# Autodesk Inventor assembly: y_carryage
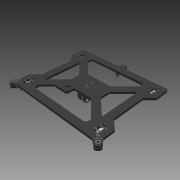
[picture p0: Inventor's stored thumbnail of the model, 180x180]
Saved by Autodesk Inventor 2014 (Build 180170000, 170)
## iProperties
Created: 2014-01-11
Part Number: y_carryage
Document SubType Name: Assembly
Designer: buben
Author: buben
## Documents named in this file (16)
- C:\Users\buben\Documents\GitHub\bacon\inventor files\assemblies\y_carryage.iam
- C:\Users\buben\Documents\GitHub\bacon\inventor files\printer parts\y_carriage.ipt
- C:\Users\buben\Documents\GitHub\bacon\inventor files\3rd party components\linear_bearing_8\Imported Components\LU8MM\LU8MM.iam
- C:\Users\buben\Documents\GitHub\bacon\inventor files\utils\washer_m5.ipt
- C:\Users\buben\Documents\GitHub\bacon\inventor files\utils\washer_m4.ipt
- C:\Users\buben\Documents\GitHub\bacon\inventor files\printer parts\y_carriage_nut_holder_a.ipt
- C:\Users\buben\Documents\GitHub\bacon\inventor files\printer parts\y_carriage_nut_holder_b.ipt
- C:\Users\buben\Documents\Inventor\Content Center Files\R2014\en-US\CSN EN 24032\ISO 4032 - M5CSN EN.ipt
- C:\Users\buben\Documents\Inventor\Content Center Files\R2014\en-US\ISO 7040\ISO 7040 - M4.ipt
- C:\Users\buben\Documents\Inventor\Content Center Files\R2014\en-US\ISO 4762(2)\ISO 4762 - M4 x 25ISO.ipt
- C:\Users\buben\Documents\GitHub\bacon\inventor files\printer parts\y_carriage_belt_mount_bed_holder.ipt
- C:\Users\buben\Documents\GitHub\bacon\inventor files\printer parts\y_carriage_belt_mount.ipt
- C:\Users\buben\Documents\Inventor\Content Center Files\R2014\en-US\ISO 4762(2)\ISO 4762 - M4 x 30ISO.ipt
- C:\Users\buben\Documents\GitHub\bacon\inventor files\utils\y_carryage_bearing_zip_tie.ipt
- C:\Users\buben\Documents\GitHub\bacon\inventor files\utils\y_carryage_nut_holder_b_zip_tie.ipt
- C:\Users\buben\Documents\GitHub\bacon\inventor files\utils\y_carryage_nut_holder_a_zip_tie.ipt
## Components (62 placed, 15 different names)
1. y_carriage:1 — Mate:4, Mate:5, Mate:6, Mate:7, Mate:8, Mate:9, Mate:10, Mate:11, Mate:12, Mate:13, Mate:14, Mate:15, Mate:16, Mate:17, Flush:1, Mate:18, Mate:19, Mate:20, Mate:21, Mate:22, Mate:23, Mate:24, Mate:25, Mate:26, Mate:27, Mate:28, Mate:29, Mate:30, Mate:31, Mate:32, Mate:33, Mate:34, Mate:35, Mate:36, Mate:37, Mate:38, Mate:39, Mate:40, Mate:41, Mate:43, Mate:45, Mate:47, Flush:2, Flush:3, Flush:4, Mate:75, Mate:76, Mate:77, Mate:78, Mate:79, Mate:80, Mate:81, Mate:102, Mate:104, Mate:105, Mate:106, Mate:108, Mate:109, Mate:111, Mate:112, Mate:114, Mate:115, Mate:117, Mate:118, Mate:120, Mate:121, Mate:123, Mate:124, Mate:126, Mate:127, Mate:128, Mate:129, Mate:130, Mate:131, Mate:132
2. LU8MM:1 [sub-assembly] — Mate:10, Mate:11, Mate:15, Mate:122, Mate:125
3. LU8MM:2 [sub-assembly] — Mate:8, Mate:9, Mate:12, Mate:116, Mate:119
4. LU8MM:3 [sub-assembly] — Mate:6, Mate:7, Mate:14, Mate:110, Mate:113
5. LU8MM:4 [sub-assembly] — Mate:4, Mate:5, Mate:13, Mate:103, Mate:107
6. CSN 02 1702 B B 5,3:1 — Mate:18, Mate:19
7. CSN 02 1702 B B 5,3:2 — Mate:20, Mate:21
8. CSN 02 1702 B B 5,3:3 — Mate:22, Mate:23
9. CSN 02 1702 B B 4,3:1 — Mate:26, Mate:27, Insert:2
10. CSN 02 1702 B B 4,3:2 — Mate:28, Mate:29, Insert:3
11. CSN 02 1702 B B 4,3:3 — Mate:30, Mate:31
12. CSN 02 1702 B B 4,3:4 — Mate:24, Mate:25, Insert:1
13. CSN 02 1702 B B 4,3:5 — Mate:34, Mate:35
14. CSN 02 1702 B B 4,3:6 — Mate:32, Mate:33
15. CSN 02 1702 B B 5,3:4 — Mate:36, Mate:37, Mate:44, Mate:62
16. CSN 02 1702 B B 5,3:5 — Mate:38, Mate:39, Mate:42, Mate:68
17. CSN 02 1702 B B 5,3:6 — Mate:40, Mate:41, Mate:46, Mate:65
18. y_carriage_nut_holder_a:1 — Mate:44, Mate:45, Flush:3, Mate:50, Mate:51, Mate:60, Mate:61
19. y_carriage_nut_holder_a:2 — Mate:46, Mate:47, Flush:2, Mate:52, Mate:53, Mate:63, Mate:64
20. y_carriage_nut_holder_b:1 — Mate:42, Mate:43, Flush:4, Mate:48, Mate:49, Mate:66, Mate:67
21. CSN 02 1702 B B 4,3:7 — Mate:48, Mate:49, Mate:58
22. CSN 02 1702 B B 4,3:8 — Mate:50, Mate:51, Mate:54
23. CSN 02 1702 B B 4,3:9 — Mate:52, Mate:53, Mate:56
24. ISO 4762 M4 x 25:1 — Insert:3, Mate:59
25. ISO 4762 M4 x 25:2 — Insert:2, Mate:57
26. ISO 4762 M4 x 25:3 — Insert:1, Mate:55
27. CSN EN 24032 M5:1 — Mate:60, Mate:61, Mate:62
28. CSN EN 24032 M5:2 — Mate:63, Mate:64, Mate:65
29. CSN EN 24032 M5:3 — Mate:66, Mate:67, Mate:68
30. DIN EN ISO 7040 M4:1 — Mate:54, Mate:55
31. DIN EN ISO 7040 M4:2 — Mate:56, Mate:57
32. DIN EN ISO 7040 M4:3 — Mate:58, Mate:59
33. y_carriage_belt_mount_bed_holder:1 — Mate:69, Mate:70, Mate:71, Mate:72, Mate:73, Mate:74, Mate:82, Mate:84
34. y_carriage_belt_mount:1 — Mate:72, Mate:73, Mate:74, Mate:76, Mate:92, Mate:93, Mate:94, Mate:95
35. y_carriage_belt_mount:2 — Mate:69, Mate:70, Mate:71, Mate:75, Mate:77, Mate:90, Mate:91, Mate:96, Mate:97
36. CSN 02 1702 B B 4,3:10 — Mate:78, Mate:81, Insert:4
37. CSN 02 1702 B B 4,3:11 — Mate:84, Mate:85, Mate:88
38. CSN 02 1702 B B 4,3:12 — Mate:82, Mate:83, Mate:86
39. CSN 02 1702 B B 4,3:13 — Mate:79, Mate:80, Insert:5
40. ISO 4762 M4 x 30:2 — Insert:4, Mate:85, Mate:89
41. ISO 4762 M4 x 30:1 — Mate:83, Mate:87, Insert:5
42. DIN EN ISO 7040 M4:4 — Mate:88, Mate:89
43. DIN EN ISO 7040 M4:5 — Mate:86, Mate:87
44. CSN 02 1702 B B 4,3:14 — Mate:93, Mate:94, Mate:100
45. CSN 02 1702 B B 4,3:15 — Mate:91, Mate:96, Insert:6
46. CSN 02 1702 B B 4,3:16 — Mate:92, Mate:95, Mate:98
47. CSN 02 1702 B B 4,3:17 — Mate:90, Mate:97, Insert:7
48. ISO 4762 M4 x 30:4 — Insert:6, Mate:99
49. ISO 4762 M4 x 30:3 — Insert:7, Mate:101
50. DIN EN ISO 7040 M4:6 — Mate:98, Mate:99
51. DIN EN ISO 7040 M4:7 — Mate:100, Mate:101
52. y_carryage_bearing_zip_tie:1 — Mate:102, Mate:103, Mate:104
53. y_carryage_bearing_zip_tie:2 — Mate:117, Mate:118, Mate:119
54. y_carryage_bearing_zip_tie:3 — Mate:111, Mate:112, Mate:113
55. y_carryage_bearing_zip_tie:4 — Mate:108, Mate:109, Mate:110
56. y_carryage_bearing_zip_tie:5 — Mate:114, Mate:115, Mate:116
57. y_carryage_bearing_zip_tie:6 — Mate:123, Mate:124, Mate:125
58. y_carryage_bearing_zip_tie:7 — Mate:105, Mate:106, Mate:107
59. y_carryage_bearing_zip_tie:8 — Mate:120, Mate:121, Mate:122
60. y_carryage_nut_holder_b_zip_tie:1 — Mate:126
61. y_carryage_nut_holder_a_zip_tie:1 — Mate:130, Mate:131, Mate:132
62. y_carryage_nut_holder_a_zip_tie:2 — Mate:127, Mate:128, Mate:129
## Relationships (140: Mate 129, Insert 7, Flush 4)
- Mate:4 (7.5 mm): y_carriage:1 ↔ LU8MM:4
- Mate:5 (7.5 mm): y_carriage:1 ↔ LU8MM:4
- Mate:6 (7.5 mm): y_carriage:1 ↔ LU8MM:3
- Mate:7 (7.5 mm): y_carriage:1 ↔ LU8MM:3
- Mate:8 (7.5 mm): y_carriage:1 ↔ LU8MM:2
- Mate:9 (7.5 mm): y_carriage:1 ↔ LU8MM:2
- Mate:10 (7.5 mm): y_carriage:1 ↔ LU8MM:1
- Mate:11 (7.5 mm): y_carriage:1 ↔ LU8MM:1
- Mate:12 (0.5 mm): y_carriage:1 ↔ LU8MM:2
- Mate:13 (0.5 mm): y_carriage:1 ↔ LU8MM:4
- Mate:14 (0.5 mm): y_carriage:1 ↔ LU8MM:3
- Mate:15 (0.5 mm): y_carriage:1 ↔ LU8MM:1
- Mate:16: y_carriage:1
- Mate:17: y_carriage:1
- Flush:1: y_carriage:1
- Mate:18: y_carriage:1 ↔ CSN 02 1702 B B 5,3:1
- Mate:19: y_carriage:1 ↔ CSN 02 1702 B B 5,3:1
- Mate:20: y_carriage:1 ↔ CSN 02 1702 B B 5,3:2
- Mate:21: y_carriage:1 ↔ CSN 02 1702 B B 5,3:2
- Mate:22: y_carriage:1 ↔ CSN 02 1702 B B 5,3:3
- Mate:23: y_carriage:1 ↔ CSN 02 1702 B B 5,3:3
- Mate:24: y_carriage:1 ↔ CSN 02 1702 B B 4,3:4
- Mate:25: y_carriage:1 ↔ CSN 02 1702 B B 4,3:4
- Mate:26: y_carriage:1 ↔ CSN 02 1702 B B 4,3:1
- Mate:27: y_carriage:1 ↔ CSN 02 1702 B B 4,3:1
- Mate:28: y_carriage:1 ↔ CSN 02 1702 B B 4,3:2
- Mate:29: y_carriage:1 ↔ CSN 02 1702 B B 4,3:2
- Mate:30: y_carriage:1 ↔ CSN 02 1702 B B 4,3:3
- Mate:31: y_carriage:1 ↔ CSN 02 1702 B B 4,3:3
- Mate:32: y_carriage:1 ↔ CSN 02 1702 B B 4,3:6
- Mate:33: y_carriage:1 ↔ CSN 02 1702 B B 4,3:6
- Mate:34: y_carriage:1 ↔ CSN 02 1702 B B 4,3:5
- Mate:35: y_carriage:1 ↔ CSN 02 1702 B B 4,3:5
- Mate:36: y_carriage:1 ↔ CSN 02 1702 B B 5,3:4
- Mate:37: y_carriage:1 ↔ CSN 02 1702 B B 5,3:4
- Mate:38: y_carriage:1 ↔ CSN 02 1702 B B 5,3:5
- Mate:39: y_carriage:1 ↔ CSN 02 1702 B B 5,3:5
- Mate:40: y_carriage:1 ↔ CSN 02 1702 B B 5,3:6
- Mate:41: y_carriage:1 ↔ CSN 02 1702 B B 5,3:6
- Mate:42: CSN 02 1702 B B 5,3:5 ↔ y_carriage_nut_holder_b:1
- Mate:43: y_carriage:1 ↔ y_carriage_nut_holder_b:1
- Mate:44: CSN 02 1702 B B 5,3:4 ↔ y_carriage_nut_holder_a:1
- Mate:45: y_carriage:1 ↔ y_carriage_nut_holder_a:1
- Mate:46: CSN 02 1702 B B 5,3:6 ↔ y_carriage_nut_holder_a:2
- Mate:47: y_carriage:1 ↔ y_carriage_nut_holder_a:2
- Flush:2: y_carriage:1 ↔ y_carriage_nut_holder_a:2
- Flush:3: y_carriage:1 ↔ y_carriage_nut_holder_a:1
- Flush:4: y_carriage:1 ↔ y_carriage_nut_holder_b:1
- Mate:48: y_carriage_nut_holder_b:1 ↔ CSN 02 1702 B B 4,3:7
- Mate:49: y_carriage_nut_holder_b:1 ↔ CSN 02 1702 B B 4,3:7
- Mate:50: y_carriage_nut_holder_a:1 ↔ CSN 02 1702 B B 4,3:8
- Mate:51: y_carriage_nut_holder_a:1 ↔ CSN 02 1702 B B 4,3:8
- Mate:52: y_carriage_nut_holder_a:2 ↔ CSN 02 1702 B B 4,3:9
- Mate:53: y_carriage_nut_holder_a:2 ↔ CSN 02 1702 B B 4,3:9
- Insert:1: CSN 02 1702 B B 4,3:4 ↔ ISO 4762 M4 x 25:3
- Insert:2: CSN 02 1702 B B 4,3:1 ↔ ISO 4762 M4 x 25:2
- Insert:3: CSN 02 1702 B B 4,3:2 ↔ ISO 4762 M4 x 25:1
- Mate:54: CSN 02 1702 B B 4,3:8 ↔ DIN EN ISO 7040 M4:1
- Mate:55: ISO 4762 M4 x 25:3 ↔ DIN EN ISO 7040 M4:1
- Mate:56: CSN 02 1702 B B 4,3:9 ↔ DIN EN ISO 7040 M4:2
- Mate:57: ISO 4762 M4 x 25:2 ↔ DIN EN ISO 7040 M4:2
- Mate:58: CSN 02 1702 B B 4,3:7 ↔ DIN EN ISO 7040 M4:3
- Mate:59: ISO 4762 M4 x 25:1 ↔ DIN EN ISO 7040 M4:3
- Mate:60: y_carriage_nut_holder_a:1 ↔ CSN EN 24032 M5:1
- Mate:61: y_carriage_nut_holder_a:1 ↔ CSN EN 24032 M5:1
- Mate:62: CSN 02 1702 B B 5,3:4 ↔ CSN EN 24032 M5:1
- Mate:63: y_carriage_nut_holder_a:2 ↔ CSN EN 24032 M5:2
- Mate:64: y_carriage_nut_holder_a:2 ↔ CSN EN 24032 M5:2
- Mate:65: CSN 02 1702 B B 5,3:6 ↔ CSN EN 24032 M5:2
- Mate:66: y_carriage_nut_holder_b:1 ↔ CSN EN 24032 M5:3
- Mate:67: y_carriage_nut_holder_b:1 ↔ CSN EN 24032 M5:3
- Mate:68: CSN 02 1702 B B 5,3:5 ↔ CSN EN 24032 M5:3
- Mate:69: y_carriage_belt_mount_bed_holder:1 ↔ y_carriage_belt_mount:2
- Mate:70: y_carriage_belt_mount_bed_holder:1 ↔ y_carriage_belt_mount:2
- Mate:71: y_carriage_belt_mount_bed_holder:1 ↔ y_carriage_belt_mount:2
- Mate:72: y_carriage_belt_mount_bed_holder:1 ↔ y_carriage_belt_mount:1
- Mate:73: y_carriage_belt_mount_bed_holder:1 ↔ y_carriage_belt_mount:1
- Mate:74: y_carriage_belt_mount_bed_holder:1 ↔ y_carriage_belt_mount:1
- Mate:75: y_carriage:1 ↔ y_carriage_belt_mount:2
- Mate:76: y_carriage:1 ↔ y_carriage_belt_mount:1
- Mate:77: y_carriage:1 ↔ y_carriage_belt_mount:2
- Mate:78: y_carriage:1 ↔ CSN 02 1702 B B 4,3:10
- Mate:79: y_carriage:1 ↔ CSN 02 1702 B B 4,3:13
- Mate:80: y_carriage:1 ↔ CSN 02 1702 B B 4,3:13
- Mate:81: y_carriage:1 ↔ CSN 02 1702 B B 4,3:10
- Insert:4: CSN 02 1702 B B 4,3:10 ↔ ISO 4762 M4 x 30:2
- Mate:82: y_carriage_belt_mount_bed_holder:1 ↔ CSN 02 1702 B B 4,3:12
- Mate:83: CSN 02 1702 B B 4,3:12 ↔ ISO 4762 M4 x 30:1
- Mate:84: y_carriage_belt_mount_bed_holder:1 ↔ CSN 02 1702 B B 4,3:11
- Mate:85: CSN 02 1702 B B 4,3:11 ↔ ISO 4762 M4 x 30:2
- Mate:86: CSN 02 1702 B B 4,3:12 ↔ DIN EN ISO 7040 M4:5
- Mate:87: ISO 4762 M4 x 30:1 ↔ DIN EN ISO 7040 M4:5
- Mate:88: CSN 02 1702 B B 4,3:11 ↔ DIN EN ISO 7040 M4:4
- Mate:89: ISO 4762 M4 x 30:2 ↔ DIN EN ISO 7040 M4:4
- Insert:5: CSN 02 1702 B B 4,3:13 ↔ ISO 4762 M4 x 30:1
- Mate:90: y_carriage_belt_mount:2 ↔ CSN 02 1702 B B 4,3:17
- Mate:91: y_carriage_belt_mount:2 ↔ CSN 02 1702 B B 4,3:15
- Mate:92: y_carriage_belt_mount:1 ↔ CSN 02 1702 B B 4,3:16
- Mate:93: y_carriage_belt_mount:1 ↔ CSN 02 1702 B B 4,3:14
- Mate:94: y_carriage_belt_mount:1 ↔ CSN 02 1702 B B 4,3:14
- Mate:95: y_carriage_belt_mount:1 ↔ CSN 02 1702 B B 4,3:16
- Mate:96: y_carriage_belt_mount:2 ↔ CSN 02 1702 B B 4,3:15
- Mate:97: y_carriage_belt_mount:2 ↔ CSN 02 1702 B B 4,3:17
- Insert:6: CSN 02 1702 B B 4,3:15 ↔ ISO 4762 M4 x 30:4
- Insert:7: CSN 02 1702 B B 4,3:17 ↔ ISO 4762 M4 x 30:3
- Mate:98: CSN 02 1702 B B 4,3:16 ↔ DIN EN ISO 7040 M4:6
- Mate:99: ISO 4762 M4 x 30:4 ↔ DIN EN ISO 7040 M4:6
- Mate:100: CSN 02 1702 B B 4,3:14 ↔ DIN EN ISO 7040 M4:7
- Mate:101: ISO 4762 M4 x 30:3 ↔ DIN EN ISO 7040 M4:7
- Mate:102: y_carriage:1 ↔ y_carryage_bearing_zip_tie:1
- Mate:103: LU8MM:4 ↔ y_carryage_bearing_zip_tie:1
- Mate:104 (5 mm): y_carriage:1 ↔ y_carryage_bearing_zip_tie:1
- Mate:105: y_carriage:1 ↔ y_carryage_bearing_zip_tie:7
- Mate:106 (5 mm): y_carriage:1 ↔ y_carryage_bearing_zip_tie:7
- Mate:107: LU8MM:4 ↔ y_carryage_bearing_zip_tie:7
- Mate:108: y_carriage:1 ↔ y_carryage_bearing_zip_tie:4
- Mate:109 (5 mm): y_carriage:1 ↔ y_carryage_bearing_zip_tie:4
- Mate:110: LU8MM:3 ↔ y_carryage_bearing_zip_tie:4
- Mate:111: y_carriage:1 ↔ y_carryage_bearing_zip_tie:3
- Mate:112 (5 mm): y_carriage:1 ↔ y_carryage_bearing_zip_tie:3
- Mate:113: LU8MM:3 ↔ y_carryage_bearing_zip_tie:3
- Mate:114: y_carriage:1 ↔ y_carryage_bearing_zip_tie:5
- Mate:115 (5 mm): y_carriage:1 ↔ y_carryage_bearing_zip_tie:5
- Mate:116: LU8MM:2 ↔ y_carryage_bearing_zip_tie:5
- Mate:117: y_carriage:1 ↔ y_carryage_bearing_zip_tie:2
- Mate:118 (5 mm): y_carriage:1 ↔ y_carryage_bearing_zip_tie:2
- Mate:119: LU8MM:2 ↔ y_carryage_bearing_zip_tie:2
- Mate:120: y_carriage:1 ↔ y_carryage_bearing_zip_tie:8
- Mate:121 (5 mm): y_carriage:1 ↔ y_carryage_bearing_zip_tie:8
- Mate:122: LU8MM:1 ↔ y_carryage_bearing_zip_tie:8
- Mate:123: y_carriage:1 ↔ y_carryage_bearing_zip_tie:6
- Mate:124 (5 mm): y_carriage:1 ↔ y_carryage_bearing_zip_tie:6
- Mate:125: LU8MM:1 ↔ y_carryage_bearing_zip_tie:6
- Mate:126: y_carriage:1 ↔ y_carryage_nut_holder_b_zip_tie:1
- Mate:127: y_carriage:1 ↔ y_carryage_nut_holder_a_zip_tie:2
- Mate:128: y_carriage:1 ↔ y_carryage_nut_holder_a_zip_tie:2
- Mate:129: y_carriage:1 ↔ y_carryage_nut_holder_a_zip_tie:2
- Mate:130: y_carriage:1 ↔ y_carryage_nut_holder_a_zip_tie:1
- Mate:131: y_carriage:1 ↔ y_carryage_nut_holder_a_zip_tie:1
- Mate:132: y_carriage:1 ↔ y_carryage_nut_holder_a_zip_tie:1
